# Autodesk Inventor assembly: Collector Arms v2.0
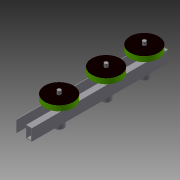
[picture p0: Inventor's stored thumbnail of the model, 180x180]
Saved by Autodesk Inventor 2015 (Build 190159000, 159)
## iProperties
Created: 2015-01-20
Part Number: Collector Arms v2.0
Document SubType Name: Assembly
Designer: chapale16
Author: chapale16
## Documents named in this file (5)
- \\lhssvr02\Homedirs\Robotics Club\CAD Model 2015\Game Components\The Tote Collector-Arms\Collector Arms v2.0.iam
- \\lhssvr02\Homedirs\Robotics Club\CAD Model 2015\Game Components\The Tote Collector-Arms\23.5 in 2 x 1 boxBeam.ipt
- \\lhssvr02\Homedirs\Robotics Club\CAD Model 2015\Game Components\The Tote Collector-Arms\23.5 sheet metal.ipt
- \\lhssvr02\Homedirs\Robotics Club\CAD Model 2015\Game Components\The Tote Collector-Arms\P60 Gear Box.ipt
- \\lhssvr02\Homedirs\Robotics Club\CAD Model 2015\Game Components\The Tote Collector-Arms\collector arm wheel.ipt
## Components (8 placed, 4 different names)
1. 23.5 in 2 x 1 boxBeam:1 — Flush:1, Mate:1, Flush:2, Mate:5, Flush:3, Mate:8, Flush:5, Flush:7, Flush:8
2. 23.5 sheet metal:1 — Mate:9, Flush:7, Flush:8
3. P60 Gear Box:2 — Flush:1, Mate:1, Flush:2, Mate:2, Mate:4, Mate:9
4. collector arm wheel:1 — Mate:2, Flush:4
5. P60 Gear Box:3 — Mate:4, Mate:5, Flush:3, Mate:7
6. collector arm wheel:2 — Flush:4, Flush:6
7. P60 Gear Box:4 — Mate:7, Mate:8, Flush:5
8. collector arm wheel:3 — Flush:6
## Relationships (17: Mate 9, Flush 8)
- Flush:1: 23.5 in 2 x 1 boxBeam:1 ↔ P60 Gear Box:2
- Mate:1: 23.5 in 2 x 1 boxBeam:1 ↔ P60 Gear Box:2
- Flush:2 (144.8308 mm): 23.5 in 2 x 1 boxBeam:1 ↔ P60 Gear Box:2
- Mate:2: P60 Gear Box:2 ↔ collector arm wheel:1
- [Mate]: P60 Gear Box:3 ↔ collector arm wheel:2
- Mate:4 (165.1 mm): P60 Gear Box:2 ↔ P60 Gear Box:3
- Mate:5: 23.5 in 2 x 1 boxBeam:1 ↔ P60 Gear Box:3
- Flush:3: 23.5 in 2 x 1 boxBeam:1 ↔ P60 Gear Box:3
- Flush:4: collector arm wheel:1 ↔ collector arm wheel:2
- [Mate]: P60 Gear Box:4 ↔ collector arm wheel:3
- Mate:7 (127 mm): P60 Gear Box:3 ↔ P60 Gear Box:4
- Mate:8: 23.5 in 2 x 1 boxBeam:1 ↔ P60 Gear Box:4
- Flush:5: 23.5 in 2 x 1 boxBeam:1 ↔ P60 Gear Box:4
- Flush:6: collector arm wheel:2 ↔ collector arm wheel:3
- Mate:9: 23.5 sheet metal:1 ↔ P60 Gear Box:2
- Flush:7: 23.5 in 2 x 1 boxBeam:1 ↔ 23.5 sheet metal:1
- Flush:8: 23.5 in 2 x 1 boxBeam:1 ↔ 23.5 sheet metal:1
## Named parameters: d4_d3 = 0 mm, d9_d3 = 0 mm
